# Autodesk Inventor assembly: Case B
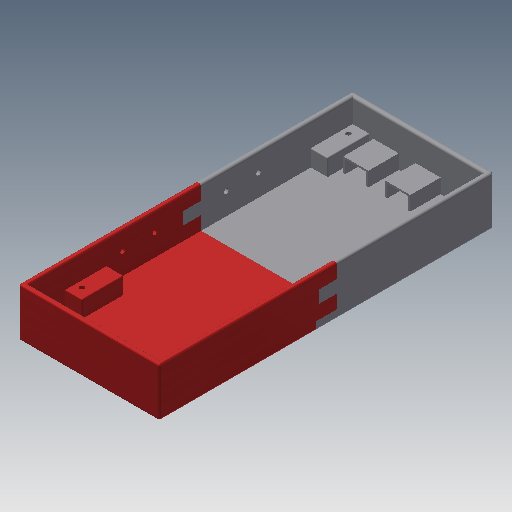
[picture p0: Inventor's stored thumbnail of the model, 512x512]
Saved by Autodesk Inventor 2019 (Build 230136000, 136)
## iProperties
Created: 2019-05-31
Part Number: Case B
Document SubType Name: Assembly
Designer: giacomo
Author: giacomo
## Documents named in this file (3)
- D:\Hobby\Inventor\Case 3Dprinted\B\Case B.iam
- D:\Hobby\Inventor\Case 3Dprinted\B\Case_B1.ipt
- D:\Hobby\Inventor\Case 3Dprinted\B\Case_B2.ipt
## Components (2 placed, 2 different names)
1. Case_B1:1 — Flush:1, Flush:2, Mate:1
2. Case_B2:1 — Flush:1, Flush:2, Mate:1
## Relationships (3: Flush 2, Mate 1)
- Flush:1: Case_B1:1 ↔ Case_B2:1
- Flush:2: Case_B1:1 ↔ Case_B2:1
- Mate:1: Case_B1:1 ↔ Case_B2:1
